# Autodesk Inventor assembly: RSX Assembly
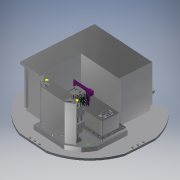
[picture p0: Inventor's stored thumbnail of the model, 180x180]
Saved by Autodesk Inventor 2017 (Build 210142000, 142)
## iProperties
Created: 2016-10-28
Part Number: RSX Assembly
Document SubType Name: Assembly
Designer: eschr_000
Author: eschr_000
## Documents named in this file (9)
- D:\UMD Near Space\star\CAD\Mechanical\CapTech\CADD\CADD\RSX Assembly\RSX Assembly.iam
- D:\UMD Near Space\star\CAD\Mechanical\CapTech\CADD\CADD\RSX Assembly\RSX Structure.ipt
- D:\UMD Near Space\star\CAD\Mechanical\CapTech\CADD\CADD\RSX Assembly\VR Camera.ipt
- D:\UMD Near Space\star\CAD\Mechanical\CapTech\CADD\CADD\RSX Assembly\VR Camera Dome.ipt
- D:\UMD Near Space\star\CAD\Mechanical\CapTech\CADD\CADD\RSX Assembly\RSX Deck.ipt
- D:\UMD Near Space\star\CAD\Mechanical\CapTech\CADD\CADD\RSX Assembly\Hermes Cube.iam
- D:\UMD Near Space\star\CAD\Mechanical\CapTech\CADD\CADD\RSX Assembly\0.25 Standoff.ipt
- D:\UMD Near Space\star\CAD\Mechanical\Full payload assembly mk 2.iam
- D:\UMD Near Space\star\CAD\Mechanical\CapTech\CTU Top.ipt
## Components (11 placed, 8 different names)
1. VR Camera:1 — Mate:14, Mate:15, Tangent:1, Tangent:2
2. VR Camera Dome:1 — Mate:14, Mate:15, Mate:53
3. RSX Deck:1 — Mate:27, Mate:28, Mate:33, Mate:36, Mate:49, Flush:2, Flush:3, Mate:52, Angle:1
4. Hermes Cube:1 [sub-assembly] — Mate:34, Mate:35, Mate:45
5. 0.25 Standoff:4 — Mate:38, Mate:43
6. Full payload assembly mk 2:1 [sub-assembly] — Mate:49, Mate:54, Mate:55
7. RSX Structure:1 — Mate:27, Mate:28, Mate:34, Mate:35, Mate:37, Mate:38, Mate:39, Mate:40, Mate:41, Mate:42, Mate:43, Mate:44, Flush:2, Flush:3, Mate:52, Tangent:1, Mate:53, Tangent:2, Mate:54, Mate:55, Mate:56, Flush:4, Flush:5
8. 0.25 Standoff:1 — Mate:40, Mate:41, Mate:45
9. 0.25 Standoff:2 — Mate:39, Mate:42
10. 0.25 Standoff:3 — Mate:37, Mate:44
11. CTU Top:1 — Mate:56, Flush:4, Flush:5
## Relationships (30: Mate 23, Flush 4, Tangent 2, Angle 1)
- Mate:14: VR Camera:1 ↔ VR Camera Dome:1
- Mate:15: VR Camera:1 ↔ VR Camera Dome:1
- Mate:27: RSX Deck:1 ↔ RSX Structure:1
- Mate:28: RSX Deck:1 ↔ RSX Structure:1
- Mate:33: RSX Deck:1
- Mate:34: Hermes Cube:1 ↔ RSX Structure:1
- Mate:35 (5.475 mm): Hermes Cube:1 ↔ RSX Structure:1
- Mate:36: RSX Deck:1
- Mate:37: RSX Structure:1 ↔ 0.25 Standoff:3
- Mate:38: 0.25 Standoff:4 ↔ RSX Structure:1
- Mate:39: RSX Structure:1 ↔ 0.25 Standoff:2
- Mate:40: RSX Structure:1 ↔ 0.25 Standoff:1
- Mate:41: RSX Structure:1 ↔ 0.25 Standoff:1
- Mate:42: RSX Structure:1 ↔ 0.25 Standoff:2
- Mate:43: 0.25 Standoff:4 ↔ RSX Structure:1
- Mate:44: RSX Structure:1 ↔ 0.25 Standoff:3
- Mate:45: Hermes Cube:1 ↔ 0.25 Standoff:1
- Mate:49: RSX Deck:1 ↔ Full payload assembly mk 2:1
- Flush:2 (66.5226 mm): RSX Deck:1 ↔ RSX Structure:1
- Flush:3 (67.7418 mm): RSX Deck:1 ↔ RSX Structure:1
- Mate:52: RSX Deck:1 ↔ RSX Structure:1
- Tangent:1: VR Camera:1 ↔ RSX Structure:1
- Mate:53 (28.575 mm): VR Camera Dome:1 ↔ RSX Structure:1
- Tangent:2: VR Camera:1 ↔ RSX Structure:1
- Mate:54 (9.525 mm): Full payload assembly mk 2:1 ↔ RSX Structure:1
- Mate:55 (12.7 mm): Full payload assembly mk 2:1 ↔ RSX Structure:1
- Angle:1 (0 deg): RSX Deck:1
- Mate:56: RSX Structure:1 ↔ CTU Top:1
- Flush:4: RSX Structure:1 ↔ CTU Top:1
- Flush:5: RSX Structure:1 ↔ CTU Top:1
